# Autodesk Inventor assembly: SCARA_montagem
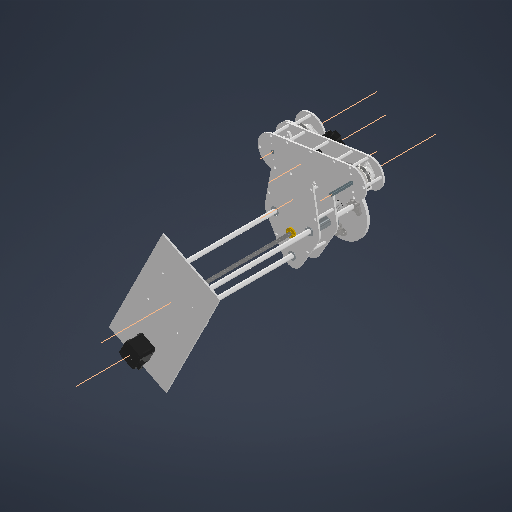
[picture p0: Inventor's stored thumbnail of the model, 512x512]
Saved by Autodesk Inventor 2025.3 (Build 293356000, 356)
## iProperties
Created: 2025-05-02
Part Number: SCARA_montagem
Document SubType Name: Assembly
Designer: Nelson
Author: Nelson
## Documents named in this file (6)
- C:\Users\Nelson\Documents\Inventor\SCARA\SCARA_montagem.iam
- C:\Users\Nelson\Documents\Inventor\SCARA\Base-Rotation.iam
- C:\Users\Nelson\Documents\Inventor\SCARA\Elo_sup.iam
- C:\Users\Nelson\Documents\Inventor\SCARA\F_TOPO.iam
- C:\Users\Nelson\Documents\Inventor\SCARA\Limit_Switch.ipt
- C:\Users\Nelson\Documents\Inventor\SCARA\Limit_Switch_L1.ipt
## Components (6 placed, 5 different names)
1. Base-Rotation:1 [sub-assembly] — Flush:1, Mate:2, Mate:3, Mate:4, Mate:5, Mate:7
2. Elo_sup:1 [sub-assembly] — Mate:1, Mate:4, Mate:8
3. F_TOPO:1 [sub-assembly] — Mate:1, Mate:2, Mate:3, Mate:5, Mate:6
4. Limit_Switch:1 — Mate:6
5. Limit_Switch_L1:1 — Mate:7
6. Limit_Switch_L1:2 — Mate:8
## Relationships (9: Mate 8, Flush 1)
- Flush:1: Base-Rotation:1
- Mate:1: Elo_sup:1 ↔ F_TOPO:1
- Mate:2: Base-Rotation:1 ↔ F_TOPO:1
- Mate:3: Base-Rotation:1 ↔ F_TOPO:1
- Mate:4: Base-Rotation:1 ↔ Elo_sup:1
- Mate:5: Base-Rotation:1 ↔ F_TOPO:1
- Mate:6: F_TOPO:1 ↔ Limit_Switch:1
- Mate:7: Base-Rotation:1 ↔ Limit_Switch_L1:1
- Mate:8: Elo_sup:1 ↔ Limit_Switch_L1:2
